# Autodesk Inventor assembly: LeapMotionAssemblyFinal
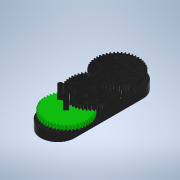
[picture p0: Inventor's stored thumbnail of the model, 180x180]
Saved by Autodesk Inventor 2022 (Build 260153000, 153)
## iProperties
Created: 2021-09-18
Part Number: LeapMotionAssemblyFinal
Document SubType Name: Assembly
Designer: marcu
Author: marcu
## Documents named in this file (6)
- C:\Users\marcu\OneDrive\Documents\Pinncale\3DPrinting\LeapMotionAssembly - Enlarged\LeapMotionAssemblyFinal.iam
- C:\Users\marcu\OneDrive\Documents\Pinncale\3DPrinting\LeapMotionAssembly - Enlarged\Board.ipt
- C:\Users\marcu\OneDrive\Documents\Pinncale\3DPrinting\LeapMotionAssembly - Enlarged\Gear2.ipt
- C:\Users\marcu\OneDrive\Documents\Pinncale\3DPrinting\LeapMotionAssembly - Enlarged\Gear1.ipt
- C:\Users\marcu\OneDrive\Documents\Pinncale\3DPrinting\LeapMotionAssembly - Enlarged\Gear2SquarePeg(2Pc).ipt
- C:\Users\marcu\OneDrive\Documents\Pinncale\3DPrinting\LeapMotionAssembly - Enlarged\Handle.ipt
## Components (7 placed, 5 different names)
1. Board:1 — Insert:1, Insert:2, Insert:3
2. Gear2:1 — Insert:1, Mate:4, Mate:5, Mate:6
3. Gear1:1 — Insert:2, Mate:1, Mate:2, Mate:3
4. Gear2SquarePeg(2Pc):1 — Mate:1, Mate:2, Mate:3
5. Gear1:2 — Insert:3, Mate:7, Mate:8, Mate:9
6. Handle:1 — Mate:4, Mate:5, Mate:6
7. Gear2SquarePeg(2Pc):2 — Mate:7, Mate:8, Mate:9
## Relationships (12: Mate 9, Insert 3)
- Insert:1: Board:1 ↔ Gear2:1
- Insert:2: Board:1 ↔ Gear1:1
- Mate:1: Gear1:1 ↔ Gear2SquarePeg(2Pc):1
- Mate:2: Gear1:1 ↔ Gear2SquarePeg(2Pc):1
- Mate:3: Gear1:1 ↔ Gear2SquarePeg(2Pc):1
- Insert:3: Board:1 ↔ Gear1:2
- Mate:4: Gear2:1 ↔ Handle:1
- Mate:5: Gear2:1 ↔ Handle:1
- Mate:6: Gear2:1 ↔ Handle:1
- Mate:7: Gear1:2 ↔ Gear2SquarePeg(2Pc):2
- Mate:8: Gear1:2 ↔ Gear2SquarePeg(2Pc):2
- Mate:9: Gear1:2 ↔ Gear2SquarePeg(2Pc):2
